# Autodesk Inventor assembly: Spool Holder Assembly
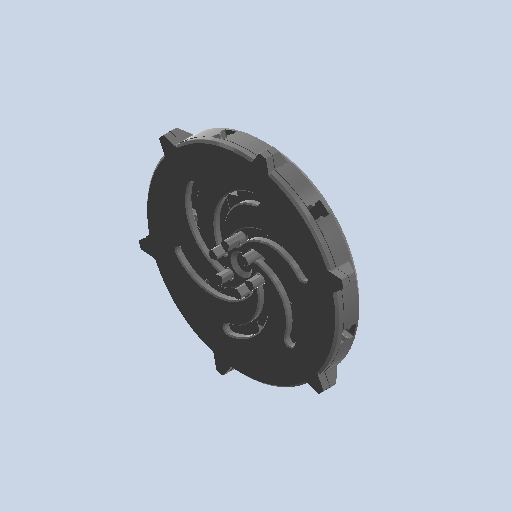
[picture p0: Inventor's stored thumbnail of the model, 512x512]
Saved by Autodesk Inventor 2024 (Build 280153000, 153)
## iProperties
Created: 2024-08-17
Part Number: Spool Holder Assembly
Document SubType Name: Assembly
Designer: Ishaan
Author: Ishaan
## Documents named in this file (7)
- E:\Projects\Axiom--IDEX-3D-Printer\CAD\05 - Spool Holder\Spool Holder Assembly.iam
- E:\Projects\Axiom--IDEX-3D-Printer\CAD\05 - Spool Holder\Spool Holder BAse.ipt
- E:\Projects\Axiom--IDEX-3D-Printer\CAD\00 - COTS Components\6704ZZ.ipt
- E:\Projects\Axiom--IDEX-3D-Printer\CAD\00 - COTS Components\6812ZZ.ipt
- E:\Projects\Axiom--IDEX-3D-Printer\CAD\05 - Spool Holder\Spool Holder Channel Rotor.ipt
- E:\Projects\Axiom--IDEX-3D-Printer\CAD\05 - Spool Holder\Spool Holder Iris Rotor.ipt
- E:\Projects\Axiom--IDEX-3D-Printer\CAD\05 - Spool Holder\Spool Holder Jaw.ipt
## Components (11 placed, 6 different names)
1. Spool Holder BAse:1 — Insert:1, Insert:2
2. 6704ZZ:1 — Insert:1, Insert:4
3. 6812ZZ:1 — Insert:2, Insert:3
4. Spool Holder Channel Rotor:1 — Insert:3, Mate:1, Mate:2, Mate:3, Mate:4, Mate:5, Mate:6, Flush:1, Mate:7, Flush:2, Mate:8, Mate:9, Flush:3
5. Spool Holder Iris Rotor:1 — Insert:4, Mate:10, Mate:11, Mate:12, Mate:13, Mate:14, Mate:15
6. Spool Holder Jaw:1 — Mate:1, Mate:2, Mate:12
7. Spool Holder Jaw:2 — Mate:3, Mate:4, Mate:11
8. Spool Holder Jaw:3 — Mate:5, Mate:6, Mate:10
9. Spool Holder Jaw:4 — Mate:9, Flush:3, Mate:13
10. Spool Holder Jaw:5 — Flush:2, Mate:8, Mate:14
11. Spool Holder Jaw:6 — Flush:1, Mate:7, Mate:15
## Relationships (22: Mate 15, Insert 4, Flush 3)
- Insert:1: Spool Holder BAse:1 ↔ 6704ZZ:1
- Insert:2: Spool Holder BAse:1 ↔ 6812ZZ:1
- Insert:3: 6812ZZ:1 ↔ Spool Holder Channel Rotor:1
- Insert:4: 6704ZZ:1 ↔ Spool Holder Iris Rotor:1
- Mate:1: Spool Holder Channel Rotor:1 ↔ Spool Holder Jaw:1
- Mate:2: Spool Holder Channel Rotor:1 ↔ Spool Holder Jaw:1
- Mate:3: Spool Holder Channel Rotor:1 ↔ Spool Holder Jaw:2
- Mate:4: Spool Holder Channel Rotor:1 ↔ Spool Holder Jaw:2
- Mate:5: Spool Holder Channel Rotor:1 ↔ Spool Holder Jaw:3
- Mate:6: Spool Holder Channel Rotor:1 ↔ Spool Holder Jaw:3
- Flush:1: Spool Holder Channel Rotor:1 ↔ Spool Holder Jaw:6
- Mate:7: Spool Holder Channel Rotor:1 ↔ Spool Holder Jaw:6
- Flush:2: Spool Holder Channel Rotor:1 ↔ Spool Holder Jaw:5
- Mate:8: Spool Holder Channel Rotor:1 ↔ Spool Holder Jaw:5
- Mate:9: Spool Holder Channel Rotor:1 ↔ Spool Holder Jaw:4
- Flush:3: Spool Holder Channel Rotor:1 ↔ Spool Holder Jaw:4
- Mate:10: Spool Holder Iris Rotor:1 ↔ Spool Holder Jaw:3
- Mate:11: Spool Holder Iris Rotor:1 ↔ Spool Holder Jaw:2
- Mate:12: Spool Holder Iris Rotor:1 ↔ Spool Holder Jaw:1
- Mate:13: Spool Holder Iris Rotor:1 ↔ Spool Holder Jaw:4
- Mate:14: Spool Holder Iris Rotor:1 ↔ Spool Holder Jaw:5
- Mate:15: Spool Holder Iris Rotor:1 ↔ Spool Holder Jaw:6
